# Autodesk Inventor assembly: MIRrightWingUnit2L
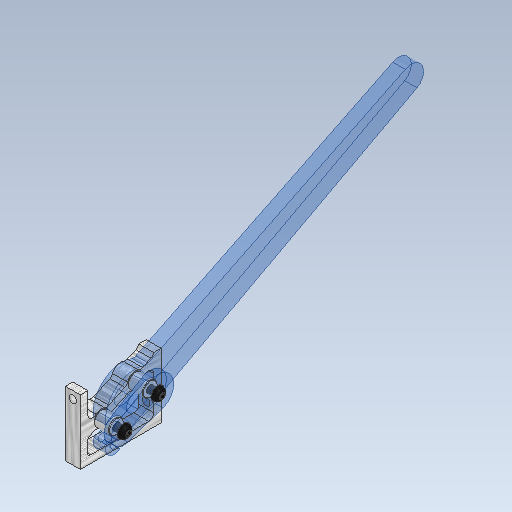
[picture p0: Inventor's stored thumbnail of the model, 512x512]
Saved by Autodesk Inventor 2020.2 (Build 242310000, 310)
## iProperties
Created: 2020-04-23
Part Number: MIRrightWingUnit2L
Document SubType Name: Assembly
Designer: aoyama
Mass: 19.7102 g
Surface Area: 89.2978 cm^2
Volume: 11.807 cm^3
Density: 1.66937 g/cm^3
Author: aoyama
## Documents named in this file (6)
- C:\Users\aoyam\Desktop\SRDC_local\Inventor\二年機\Geminiβ\翼\MIRrightWingUnit2L.iam
- C:\Users\aoyam\Desktop\SRDC_local\Inventor\二年機\Geminiβ\翼\MIRrightWing2台座.ipt
- C:\Users\aoyam\Desktop\SRDC_local\Inventor\二年機\Geminiβ\翼\MIRrightWing2.ipt
- C:\Users\aoyam\Desktop\SRDC_local\Inventor\二年機\Geminiβ\翼\MIRrightWing抑え2.ipt
- C:\Users\aoyam\Desktop\SRDC_local\Inventor\二年機\Geminiβ\汎用部品\MIRrightスペーサー中空M3L6アルミ.ipt
- C:\Users\aoyam\Desktop\SRDC_local\Inventor\二年機\Geminiβ\汎用部品\MIRrightネジボタンM3L15.ipt
## Components (7 placed, 5 different names)
1. MIRrightWing2台座:1 — 挿入:3, 挿入:4
2. MIRrightWing2:1 — 挿入:9, 挿入:10
3. MIRrightWing抑え2:1 — 挿入:5, 挿入:7, 挿入:6, 挿入:8
4. MIRrightスペーサー中空M3L6アルミ:1 — 挿入:5, 挿入:3, 挿入:10
5. MIRrightスペーサー中空M3L6アルミ:2 — 挿入:4, 挿入:8, 挿入:9
6. MIRrightネジボタンM3L15:1 — 挿入:7
7. MIRrightネジボタンM3L15:2 — 挿入:6
## Relationships (8: Insert 8)
- 挿入:5 [Insert]: MIRrightWing抑え2:1 ↔ MIRrightスペーサー中空M3L6アルミ:1
- 挿入:3 [Insert]: MIRrightWing2台座:1 ↔ MIRrightスペーサー中空M3L6アルミ:1
- 挿入:4 [Insert]: MIRrightWing2台座:1 ↔ MIRrightスペーサー中空M3L6アルミ:2
- 挿入:7 [Insert]: MIRrightWing抑え2:1 ↔ MIRrightネジボタンM3L15:1
- 挿入:6 [Insert]: MIRrightWing抑え2:1 ↔ MIRrightネジボタンM3L15:2
- 挿入:8 [Insert]: MIRrightWing抑え2:1 ↔ MIRrightスペーサー中空M3L6アルミ:2
- 挿入:9 [Insert]: MIRrightWing2:1 ↔ MIRrightスペーサー中空M3L6アルミ:2
- 挿入:10 [Insert]: MIRrightWing2:1 ↔ MIRrightスペーサー中空M3L6アルミ:1
